# Autodesk Inventor assembly: water_boat
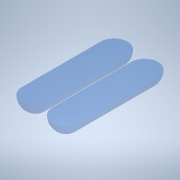
[picture p0: Inventor's stored thumbnail of the model, 180x180]
Saved by Autodesk Inventor 2020.2 (Build 242310000, 310)
## iProperties
Created: 2020-03-22
Part Number: water_boat
Document SubType Name: Assembly
Designer: agmle
Mass: 29566 g
Surface Area: 9466.62 cm^2
Volume: 29616.3 cm^3
Density: 0.9983 g/cm^3
Author: agmle
## Documents named in this file (2)
- M:\documents\Inventor\AutoBuoy\hull\water_boat.iam
- M:\documents\Inventor\AutoBuoy\hull\water_hull.ipt
## Components (2 placed, 1 different names)
1. water_hull:1 — Flush:1, Flush:2
2. water_hull:2 — Flush:2
## Relationships (2: Flush 2)
- Flush:1: water_hull:1
- Flush:2: water_hull:1 ↔ water_hull:2
